# Autodesk Inventor assembly: Prototipo2
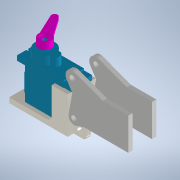
[picture p0: Inventor's stored thumbnail of the model, 180x180]
Saved by Autodesk Inventor 2020 (Build 240168000, 168)
## iProperties
Created: 2021-08-13
Part Number: Prototipo2
Document SubType Name: Assembly
Designer: chalo
Author: chalo
## Documents named in this file (4)
- C:\Users\chalo\OneDrive\Documents\GitHub\Interfaces-Biomedicas-2021\Gonzalo Palarea\Inventor\tipo2\Prototipo2.iam
- C:\Users\chalo\OneDrive\Documents\GitHub\Interfaces-Biomedicas-2021\Gonzalo Palarea\Inventor\stls\Base_v2.ipt
- C:\Users\chalo\OneDrive\Documents\GitHub\Interfaces-Biomedicas-2021\Gonzalo Palarea\Inventor\servoconbrazo.iam
- C:\Users\chalo\OneDrive\Documents\GitHub\Interfaces-Biomedicas-2021\Gonzalo Palarea\Inventor\tipo2\Metacarpo.ipt
## Components (3 placed, 3 different names)
1. Base_v2:1 — Mate:1, Angle:1, Insert:1, Flush:1, Flush:2
2. servoconbrazo:1 [sub-assembly] — Mate:1, Angle:1, Insert:1
3. Metacarpo:1 — Flush:1, Flush:2
## Relationships (5: Flush 2, Mate 1, Angle 1, Insert 1)
- Mate:1: Base_v2:1 ↔ servoconbrazo:1
- Angle:1 (0 deg): Base_v2:1 ↔ servoconbrazo:1
- Insert:1: Base_v2:1 ↔ servoconbrazo:1
- Flush:1: Base_v2:1 ↔ Metacarpo:1
- Flush:2: Base_v2:1 ↔ Metacarpo:1
